# Autodesk Inventor assembly: Noodle Sucker
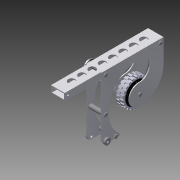
[picture p0: Inventor's stored thumbnail of the model, 180x180]
Saved by Autodesk Inventor 2015 (Build 190159000, 159)
## iProperties
Created: 2015-02-22
Part Number: Noodle Sucker
Document SubType Name: Assembly
Designer: Jarod
Author: Jarod
## Documents named in this file (13)
- D:\Robotics\FRC\2015\CAD\Robot\Noodle Sucker\Noodle Sucker.iam
- D:\Robotics\FRC\2015\CAD\Robot\Noodle Sucker\2x1 mounting.ipt
- D:\Robotics\FRC\2015\CAD\Robot\Noodle Sucker\Imported Components\4 in HiGrip Wheel\4 in HiGrip Wheel.iam
- D:\Robotics\FRC\2015\CAD\Robot\Noodle Sucker\Imported Components\VEXpro-VersaPlanetary-2stage-with-BAG\VEXpro-VersaPlanetary-2stage-with-BAG.iam
- D:\Robotics\FRC\2015\CAD\Robot\Noodle Sucker\Imported Components\hub hex 0.5in\hub hex 0.5in.ipt
- D:\Robotics\FRC\2015\CAD\Robot\Noodle Sucker\rail.ipt
- D:\Robotics\FRC\2015\CAD\Robot\Noodle Sucker\Imported Components\0.5 Hex Shaft Collar\0.5 Hex Shaft Collar.ipt
- D:\Robotics\FRC\2015\CAD\Robot\Noodle Sucker\washer.ipt
- D:\Robotics\FRC\2015\CAD\Robot\Noodle Sucker\bolt.ipt
- D:\Robotics\FRC\2015\CAD\Robot\Noodle Sucker\support bolt.ipt
- D:\Robotics\FRC\2015\CAD\Robot\Noodle Sucker\spacer.ipt
- D:\Robotics\FRC\2015\CAD\Robot\Noodle Sucker\bearing wheel.ipt
- D:\Robotics\FRC\2015\CAD\Robot\Noodle Sucker\rail gearbox mounting.ipt
## Components (17 placed, 12 different names)
1. rail:1 — Mate:7, Flush:1, Flush:2, Mate:22, Mate:23, Mate:24, Mate:25, Mate:26, Mate:27, Mate:28, Mate:29, Mate:31, Mate:33, Mate:34, Mate:35, Mate:40
2. rail gearbox mounting:1 — Mate:43, Flush:3, Flush:4, Mate:44, Mate:45, Mate:46, Mate:47, Mate:48, Mate:49
3. 2x1 mounting:1 — Mate:7, Flush:1, Flush:2, Mate:43, Flush:3, Flush:4
4. 4 in HiGrip Wheel:1 [sub-assembly] — Mate:4, Mate:5, Mate:6, Mate:18
5. VEXpro-VersaPlanetary-2stage-with-BAG:1 [sub-assembly] — Mate:6, Mate:15, Mate:19, Mate:20, Mate:46, Mate:47, Mate:48
6. hub hex 0.5in:1 — Mate:4, Mate:5, Mate:16
7. 0.5 Hex Shaft Collar:1 — Mate:15, Mate:16, Mate:49
8. washer:1 — Mate:18, Mate:19
9. bolt:1 — Mate:20, Mate:40
10. support bolt:1 — Mate:22, Mate:23, Mate:30
11. support bolt:2 — Mate:24, Mate:25, Mate:32
12. support bolt:3 — Mate:26, Mate:28
13. support bolt:4 — Mate:27, Mate:29
14. spacer:1 — Mate:30, Mate:31
15. spacer:2 — Mate:32, Mate:33
16. bearing wheel:1 — Mate:34, Mate:35
17. bearing wheel:2 — Mate:44, Mate:45
## Relationships (35: Mate 31, Flush 4)
- Mate:4: 4 in HiGrip Wheel:1 ↔ hub hex 0.5in:1
- Mate:5: 4 in HiGrip Wheel:1 ↔ hub hex 0.5in:1
- Mate:6: 4 in HiGrip Wheel:1 ↔ VEXpro-VersaPlanetary-2stage-with-BAG:1
- Mate:7: rail:1 ↔ 2x1 mounting:1
- Flush:1: rail:1 ↔ 2x1 mounting:1
- Flush:2: rail:1 ↔ 2x1 mounting:1
- Mate:15: VEXpro-VersaPlanetary-2stage-with-BAG:1 ↔ 0.5 Hex Shaft Collar:1
- Mate:16: hub hex 0.5in:1 ↔ 0.5 Hex Shaft Collar:1
- Mate:18: 4 in HiGrip Wheel:1 ↔ washer:1
- Mate:19: VEXpro-VersaPlanetary-2stage-with-BAG:1 ↔ washer:1
- Mate:20: VEXpro-VersaPlanetary-2stage-with-BAG:1 ↔ bolt:1
- Mate:22: rail:1 ↔ support bolt:1
- Mate:23: rail:1 ↔ support bolt:1
- Mate:24: rail:1 ↔ support bolt:2
- Mate:25: rail:1 ↔ support bolt:2
- Mate:26: rail:1 ↔ support bolt:3
- Mate:27: rail:1 ↔ support bolt:4
- Mate:28: rail:1 ↔ support bolt:3
- Mate:29: rail:1 ↔ support bolt:4
- Mate:30: support bolt:1 ↔ spacer:1
- Mate:31: rail:1 ↔ spacer:1
- Mate:32: support bolt:2 ↔ spacer:2
- Mate:33: rail:1 ↔ spacer:2
- Mate:34: rail:1 ↔ bearing wheel:1
- Mate:35: rail:1 ↔ bearing wheel:1
- Mate:40: rail:1 ↔ bolt:1
- Mate:43: rail gearbox mounting:1 ↔ 2x1 mounting:1
- Flush:3: rail gearbox mounting:1 ↔ 2x1 mounting:1
- Flush:4: rail gearbox mounting:1 ↔ 2x1 mounting:1
- Mate:44: rail gearbox mounting:1 ↔ bearing wheel:2
- Mate:45: rail gearbox mounting:1 ↔ bearing wheel:2
- Mate:46: rail gearbox mounting:1 ↔ VEXpro-VersaPlanetary-2stage-with-BAG:1
- Mate:47: rail gearbox mounting:1 ↔ VEXpro-VersaPlanetary-2stage-with-BAG:1
- Mate:48: rail gearbox mounting:1 ↔ VEXpro-VersaPlanetary-2stage-with-BAG:1
- Mate:49 (1.5875 mm): rail gearbox mounting:1 ↔ 0.5 Hex Shaft Collar:1
